# Autodesk Inventor assembly: Assembly
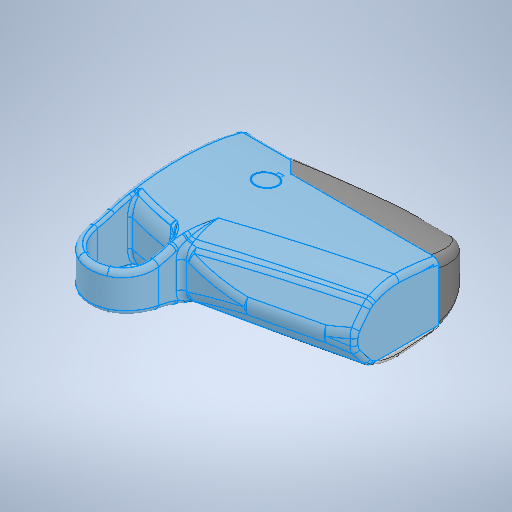
[picture p0: Inventor's stored thumbnail of the model, 512x512]
Saved by Autodesk Inventor 2025.2 (Build 292293000, 293)
## iProperties
Created: 2024-12-22
Part Number: Assembly
Document SubType Name: Assembly
Designer: naka6
Author: naka6
## Documents named in this file (18)
- C:\Users\naka6\OneDrive\ドキュメント\New Controller\Hardware\Assembly.iam
- C:\Users\naka6\OneDrive\ドキュメント\New Controller\Hardware\Body_compleat01.ipt
- C:\Users\naka6\OneDrive\ドキュメント\New Controller\Hardware\arduino-nano-33-ble-1.snapshot.2\Nano33BLE\Nano33BLE\Nano33BLE.ipt
- C:\Users\naka6\OneDrive\ドキュメント\New Controller\Hardware\bluetooth-module-hc-05-1.snapshot.4\Bluetooth Module HC-05\STEP\Bluetooth Module HC-05\Bluetooth Module HC-05.ipt
- C:\Users\naka6\OneDrive\ドキュメント\New Controller\Hardware\cad-8-pin-header-1.snapshot.2\1_Dupont_Stiftleiste v6\1_Dupont_Stiftleiste v6.ipt
- C:\Users\naka6\OneDrive\ドキュメント\New Controller\Hardware\male-header-pins-1.snapshot.11\Male Header Pin Config\Male Header Pin Config.ipt
- C:\Users\naka6\OneDrive\ドキュメント\New Controller\Hardware\Cursuit\Cuicuit\Cuicuit\Cuicuit.ipt
- C:\Users\naka6\OneDrive\ドキュメント\New Controller\Hardware\Part1.ipt
- C:\Users\naka6\OneDrive\ドキュメント\Inventor\AAA Battery.ipt
- C:\Users\naka6\OneDrive\ドキュメント\New Controller\Hardware\mini vibrator.ipt
- C:\Users\naka6\OneDrive\ドキュメント\New Controller\Hardware\switch.ipt
- C:\Users\naka6\OneDrive\ドキュメント\New Controller\Hardware\Body_compleat02.ipt
- C:\Users\naka6\OneDrive\ドキュメント\New Controller\Hardware\Part2.ipt
- C:\Users\naka6\OneDrive\ドキュメント\New Controller\Hardware\bend_sensor.ipt
- C:\Users\naka6\OneDrive\ドキュメント\New Controller\Hardware\Part3.ipt
- C:\Users\naka6\OneDrive\ドキュメント\New Controller\Hardware\cable.ipt
- C:\Users\naka6\OneDrive\ドキュメント\New Controller\Hardware\cable - コピー.ipt
- C:\Users\naka6\OneDrive\ドキュメント\New Controller\Hardware\floar.ipt
## Components (18 placed, 17 different names)
1. Body_compleat01:1 — 角度:1, 角度:2, フラッシュ:7, 角度:3, 角度:4, 角度:5, 角度:6, 角度:7, フラッシュ:8, フラッシュ:9, メイト:11, フラッシュ:10, メイト:12, フラッシュ:11, フラッシュ:12, メイト:13, メイト:14, 正接:1, フラッシュ:13, メイト:15
2. Nano33BLE:1 — メイト:4, フラッシュ:1, フラッシュ:2, 角度:1, フラッシュ:9
3. Bluetooth Module HC-05:1 — メイト:6, メイト:7, メイト:8
4. 1_Dupont_Stiftleiste v6:1 — メイト:1, メイト:2, メイト:3, メイト:5, フラッシュ:3, フラッシュ:4
5. Male Header Pin Config:1 — メイト:1, メイト:2, メイト:3, メイト:4, フラッシュ:1, フラッシュ:2
6. Cuicuit:1 — メイト:5, フラッシュ:3, フラッシュ:4, 角度:2, メイト:6, メイト:7, メイト:8, フラッシュ:5, メイト:9, フラッシュ:6, メイト:11, フラッシュ:10
7. Part1:1 — フラッシュ:5, メイト:9, フラッシュ:6
8. AAA Battery:1 — 角度:3
9. AAA Battery:2 — 角度:4
10. mini vibrator:1 — 角度:5, メイト:15, メイト:16, 正接:2, 挿入:2, 挿入:3
11. switch:1 — 角度:6, 角度:7, フラッシュ:8
12. Body_compleat02:1 — メイト:12, フラッシュ:11, フラッシュ:12
13. Part2:1 — メイト:13
14. bend_sensor:1 — メイト:14, 正接:1, フラッシュ:13
15. Part3:1 — メイト:16, 正接:2
16. cable:1 — 挿入:3
17. cable - コピー:1 — 挿入:2
18. floar:1
## Relationships (39: Mate 15, Flush 13, Angle 7, Tangent 2, Insert 2)
- メイト:1 [Mate]: 1_Dupont_Stiftleiste v6:1 ↔ Male Header Pin Config:1
- メイト:2 [Mate]: 1_Dupont_Stiftleiste v6:1 ↔ Male Header Pin Config:1
- メイト:3 [Mate]: 1_Dupont_Stiftleiste v6:1 ↔ Male Header Pin Config:1
- メイト:4 [Mate]: Nano33BLE:1 ↔ Male Header Pin Config:1
- フラッシュ:1 [Flush]: Nano33BLE:1 ↔ Male Header Pin Config:1
- フラッシュ:2 [Flush] (2.54 mm): Nano33BLE:1 ↔ Male Header Pin Config:1
- メイト:5 [Mate]: 1_Dupont_Stiftleiste v6:1 ↔ Cuicuit:1
- フラッシュ:3 [Flush] (0.3048 mm): 1_Dupont_Stiftleiste v6:1 ↔ Cuicuit:1
- フラッシュ:4 [Flush] (2.54 mm): 1_Dupont_Stiftleiste v6:1 ↔ Cuicuit:1
- 角度:1 [Angle] (0 deg): Body_compleat01:1 ↔ Nano33BLE:1
- 角度:2 [Angle] (0 deg): Body_compleat01:1 ↔ Cuicuit:1
- メイト:6 [Mate]: Bluetooth Module HC-05:1 ↔ Cuicuit:1
- メイト:7 [Mate] (0.0508 mm): Bluetooth Module HC-05:1 ↔ Cuicuit:1
- メイト:8 [Mate] (0.0508 mm): Bluetooth Module HC-05:1 ↔ Cuicuit:1
- フラッシュ:5 [Flush]: Cuicuit:1 ↔ Part1:1
- メイト:9 [Mate]: Cuicuit:1 ↔ Part1:1
- フラッシュ:6 [Flush] (0.3 mm): Cuicuit:1 ↔ Part1:1
- フラッシュ:7 [Flush]: Body_compleat01:1
- 角度:3 [Angle] (0 deg): Body_compleat01:1 ↔ AAA Battery:1
- 角度:4 [Angle] (0 deg): Body_compleat01:1 ↔ AAA Battery:2
- 角度:5 [Angle] (180 deg): Body_compleat01:1 ↔ mini vibrator:1
- 角度:6 [Angle] (0 deg): Body_compleat01:1 ↔ switch:1
- 角度:7 [Angle] (0 deg): Body_compleat01:1 ↔ switch:1
- フラッシュ:8 [Flush] (2.2 mm): Body_compleat01:1 ↔ switch:1
- フラッシュ:9 [Flush] (1.4 mm): Body_compleat01:1 ↔ Nano33BLE:1
- メイト:11 [Mate] (2.1 mm): Body_compleat01:1 ↔ Cuicuit:1
- フラッシュ:10 [Flush] (2.8 mm): Body_compleat01:1 ↔ Cuicuit:1
- メイト:12 [Mate]: Body_compleat01:1 ↔ Body_compleat02:1
- フラッシュ:11 [Flush]: Body_compleat01:1 ↔ Body_compleat02:1
- フラッシュ:12 [Flush]: Body_compleat01:1 ↔ Body_compleat02:1
- メイト:13 [Mate]: Body_compleat01:1 ↔ Part2:1
- メイト:14 [Mate]: Body_compleat01:1 ↔ bend_sensor:1
- 正接:1 [Tangent]: Body_compleat01:1 ↔ bend_sensor:1
- フラッシュ:13 [Flush] (7.5 mm): Body_compleat01:1 ↔ bend_sensor:1
- メイト:15 [Mate]: Body_compleat01:1 ↔ mini vibrator:1
- メイト:16 [Mate]: mini vibrator:1 ↔ Part3:1
- 正接:2 [Tangent] (-0.5 mm): mini vibrator:1 ↔ Part3:1
- 挿入:2 [Insert]: mini vibrator:1 ↔ cable - コピー:1
- 挿入:3 [Insert]: mini vibrator:1 ↔ cable:1
